# Autodesk Inventor assembly: WheelAssembly
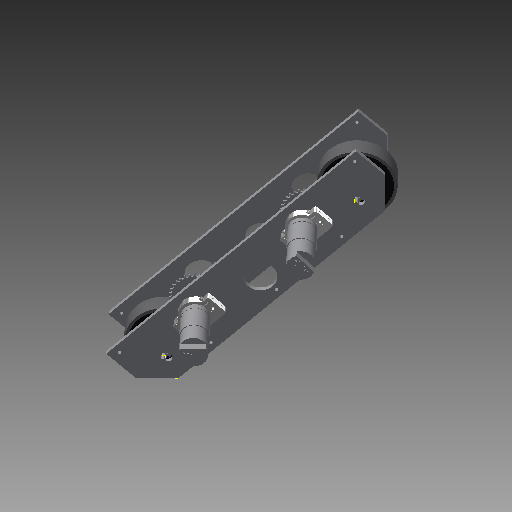
[picture p0: Inventor's stored thumbnail of the model, 512x512]
Saved by Autodesk Inventor 2017 (Build 210142000, 142)
## iProperties
Created: 2016-09-10
Part Number: WheelAssembly
Document SubType Name: Assembly
Designer: RoboticsUser
Author: RoboticsUser
## Documents named in this file (9)
- C:\Robotics\CAD\2016-17_CAD\DriveTrain\WheelAssemblyLeft.iam
- C:\Robotics\CAD\2015-16_CAD\custom cad parts\am-2648_4inWheel8mmHub.ipt
- C:\Robotics\CAD\COTSParts\Actobotics\545 parts\545456PatternAdapter.77in.625in.ipt
- C:\Robotics\CAD\COTSParts\Actobotics\615 parts\615102Sprocket.5inBore.25inPitch16Teeth.ipt
- C:\Robotics\CAD\COTSParts\Actobotics\634 parts\634080.25inDShaft4inLong.ipt
- C:\Robotics\CAD\COTSParts\Motors\Andymark 2964  NeveRest 40 Motor.ipt
- C:\Robotics\CAD\COTSParts\Actobotics\615 parts\615114Sprocket.5inBore.25inPitch32Teeth.ipt
- C:\Robotics\CAD\COTSParts\Tetrix\tetrix-motor-mounts-1.snapshot.1\Tetrex 2pc motor mount.ipt
- C:\Robotics\CAD\2016-17_CAD\DriveTrain\DrainTrainPlate1.1Inside.iam
## Components (22 placed, 8 different names)
1. am-2648_4inWheel8mmHub:2 — Insert:71, Insert:77
2. 545456PatternAdapter.77in.625in:2 — Insert:72
3. 615102Sprocket.5inBore.25inPitch16Teeth:4 — Insert:44, Insert:77
4. 634080.25inDShaft4inLong:2 — Insert:70, Insert:78
5. am-2648_4inWheel8mmHub:3 — Insert:73, Insert:74
6. 545456PatternAdapter.77in.625in:6 — Insert:75
7. 615102Sprocket.5inBore.25inPitch16Teeth:5 — Insert:54, Angle:1
8. 634080.25inDShaft4inLong:3 — Insert:66, Insert:79
9. Andymark 2964  NeveRest 40 Motor:2 — Insert:27, Insert:60
10. 545456PatternAdapter.77in.625in:8 — Insert:61
11. 615114Sprocket.5inBore.25inPitch32Teeth:2 — Insert:60, Insert:61
12. 615114Sprocket.5inBore.25inPitch32Teeth:3 — Insert:58, Insert:59
13. 545456PatternAdapter.77in.625in:9 — Insert:59
14. Andymark 2964  NeveRest 40 Motor:3 — Insert:28, Insert:58
15. Tetrex 2pc motor mount:1 — Insert:27, Insert:62, Insert:63
16. Tetrex 2pc motor mount:2 — Insert:28, Insert:64, Insert:65
17. DrainTrainPlate1.1Inside:1 [sub-assembly] — Insert:62, Insert:63, Insert:64, Insert:65, Insert:66, Insert:67, Insert:70, Insert:76
18. DrainTrainPlate1.1Inside:2 [sub-assembly] — Insert:78, Insert:79
19. 545456PatternAdapter.77in.625in:10 — Insert:44, Insert:76
20. 545456PatternAdapter.77in.625in:12 — Insert:71, Insert:72
21. 545456PatternAdapter.77in.625in:13 — Insert:74, Insert:75
22. 545456PatternAdapter.77in.625in:11 — Insert:54, Insert:67, Mate:2, Insert:73
## Relationships (26: Insert 24, Mate 1, Angle 1)
- Insert:27 (6.35 mm): Andymark 2964  NeveRest 40 Motor:2 ↔ Tetrex 2pc motor mount:1
- Insert:28 (6.35 mm): Andymark 2964  NeveRest 40 Motor:3 ↔ Tetrex 2pc motor mount:2
- Insert:44: 615102Sprocket.5inBore.25inPitch16Teeth:4 ↔ 545456PatternAdapter.77in.625in:10
- Insert:54: 615102Sprocket.5inBore.25inPitch16Teeth:5 ↔ 545456PatternAdapter.77in.625in:11
- Insert:58 (16.0274 mm): 615114Sprocket.5inBore.25inPitch32Teeth:3 ↔ Andymark 2964  NeveRest 40 Motor:3
- Insert:59: 615114Sprocket.5inBore.25inPitch32Teeth:3 ↔ 545456PatternAdapter.77in.625in:9
- Insert:60 (16.0274 mm): Andymark 2964  NeveRest 40 Motor:2 ↔ 615114Sprocket.5inBore.25inPitch32Teeth:2
- Insert:61: 545456PatternAdapter.77in.625in:8 ↔ 615114Sprocket.5inBore.25inPitch32Teeth:2
- Insert:62: Tetrex 2pc motor mount:1 ↔ DrainTrainPlate1.1Inside:1
- Insert:63: Tetrex 2pc motor mount:1 ↔ DrainTrainPlate1.1Inside:1
- Insert:64: Tetrex 2pc motor mount:2 ↔ DrainTrainPlate1.1Inside:1
- Insert:65: Tetrex 2pc motor mount:2 ↔ DrainTrainPlate1.1Inside:1
- Insert:66 (-6.35 mm): 634080.25inDShaft4inLong:3 ↔ DrainTrainPlate1.1Inside:1
- Insert:67 (3.175 mm): DrainTrainPlate1.1Inside:1 ↔ 545456PatternAdapter.77in.625in:11
- Mate:2: 545456PatternAdapter.77in.625in:11
- Angle:1 (0 deg): 615102Sprocket.5inBore.25inPitch16Teeth:5
- Insert:70 (-6.35 mm): 634080.25inDShaft4inLong:2 ↔ DrainTrainPlate1.1Inside:1
- Insert:71: am-2648_4inWheel8mmHub:2 ↔ 545456PatternAdapter.77in.625in:12
- Insert:72: 545456PatternAdapter.77in.625in:2 ↔ 545456PatternAdapter.77in.625in:12
- Insert:73 (9.525 mm): am-2648_4inWheel8mmHub:3 ↔ 545456PatternAdapter.77in.625in:11
- Insert:74: am-2648_4inWheel8mmHub:3 ↔ 545456PatternAdapter.77in.625in:13
- Insert:75: 545456PatternAdapter.77in.625in:6 ↔ 545456PatternAdapter.77in.625in:13
- Insert:76 (3.175 mm): DrainTrainPlate1.1Inside:1 ↔ 545456PatternAdapter.77in.625in:10
- Insert:77 (9.525 mm): am-2648_4inWheel8mmHub:2 ↔ 615102Sprocket.5inBore.25inPitch16Teeth:4
- Insert:78 (-19.05 mm): 634080.25inDShaft4inLong:2 ↔ DrainTrainPlate1.1Inside:2
- Insert:79 (-19.05 mm): 634080.25inDShaft4inLong:3 ↔ DrainTrainPlate1.1Inside:2
